# Autodesk Inventor assembly: SP40-10 MARCO HOJA CORREDERA 1131x695
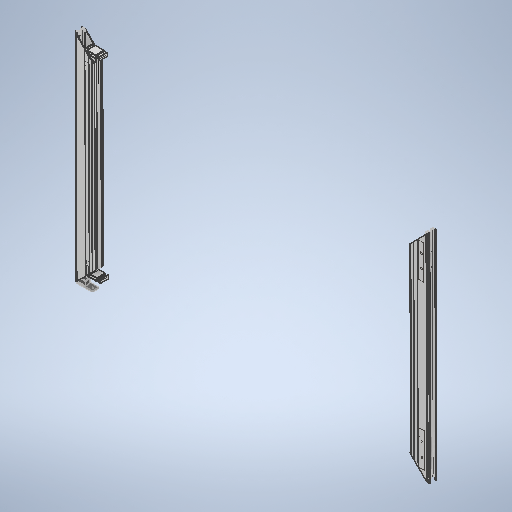
[picture p0: Inventor's stored thumbnail of the model, 512x512]
Saved by Autodesk Inventor 2025 (Build 290162000, 162)
## iProperties
Created: 2026-02-17
Part Number: SP40-10 MARCO HOJA CORREDERA 1131x695
Document SubType Name: Assembly
Designer: Frank
Author: Frank
## Documents named in this file (29)
- C:\Users\Frank\OneDrive\CARPINTERIA ALUMINIO\PUERTAS Y VENTANAS\VENTANAS\VENTANAS\ENSAMBLES\HOJA CORREDERA SP40-10 EXT 1400x1200 - DERECHA TRASERA.iam
- C:\Users\Frank\OneDrive\CARPINTERIA ALUMINIO\PUERTAS Y VENTANAS\VENTANAS\VENTANAS\PIEZAS\HOJA CORREDERA SP40-10 EXT 1400x1200\SP40-10 HOJA CORREDERA 1131 mm.ipt
- C:\Users\Frank\OneDrive\CARPINTERIA ALUMINIO\PUERTAS Y VENTANAS\VENTANAS\VENTANAS\PIEZAS\HOJA CORREDERA SP40-10 EXT 1400x1200\SP40-10 HOJA CORREDERA 695 mm.ipt
- C:\Users\Frank\OneDrive\CARPINTERIA ALUMINIO\PUERTAS Y VENTANAS\VENTANAS\VENTANAS\PIEZAS\HOJA CORREDERA SP40-10 EXT 1400x1200\SP40-10 HOJA CORREDERA 695 mm_MIR.ipt
- C:\Users\Frank\OneDrive\CARPINTERIA ALUMINIO\PUERTAS Y VENTANAS\VENTANAS\VENTANAS\PIEZAS\HOJA CORREDERA SP40-10 EXT 1400x1200\SP40-10 HOJA CORREDERA 1131 mm_MIR.ipt
- C:\Users\Frank\OneDrive\CARPINTERIA ALUMINIO\PUERTAS Y VENTANAS\VENTANAS\VENTANAS\PIEZAS\HOJA CORREDERA SP40-10 EXT 1400x1200\BRA-12 ESCUADRA UNIÓN 45 10 mm.ipt
- C:\Users\Frank\OneDrive\CARPINTERIA ALUMINIO\PUERTAS Y VENTANAS\VENTANAS\VENTANAS\PIEZAS\HOJA CORREDERA SP40-10 EXT 1400x1200\BRA-12 ESCUADRA UNIÓN 45 10 mm_MIR.ipt
- C:\Users\Frank\OneDrive\CARPINTERIA ALUMINIO\PUERTAS Y VENTANAS\VENTANAS\VENTANAS\PIEZAS\HOJA CORREDERA SP40-10 EXT 1400x1200\BRA-12 ESCUADRA UNIÓN 45 10 mm_MIR1.ipt
- C:\Users\Frank\OneDrive\CARPINTERIA ALUMINIO\PUERTAS Y VENTANAS\VENTANAS\VENTANAS\PIEZAS\HOJA CORREDERA SP40-10 EXT 1400x1200\BRA-12 ESCUADRA UNIÓN 45 10 mm_MIR2.ipt
- C:\Users\Frank\OneDrive\CARPINTERIA ALUMINIO\PUERTAS Y VENTANAS\VENTANAS\VENTANAS\PIEZAS\HOJA CORREDERA SP40-10 EXT 1400x1200\SP40-10 JUNTA INT 1025 mm.ipt
- C:\Users\Frank\OneDrive\CARPINTERIA ALUMINIO\PUERTAS Y VENTANAS\VENTANAS\VENTANAS\PIEZAS\HOJA CORREDERA SP40-10 EXT 1400x1200\SP40-10 JUNTA INT 1025 mm_MIR.ipt
- C:\Users\Frank\OneDrive\CARPINTERIA ALUMINIO\PUERTAS Y VENTANAS\VENTANAS\VENTANAS\PIEZAS\HOJA CORREDERA SP40-10 EXT 1400x1200\SP40-10 JUNTA INT 589 mm.ipt
- C:\Users\Frank\OneDrive\CARPINTERIA ALUMINIO\PUERTAS Y VENTANAS\VENTANAS\VENTANAS\PIEZAS\HOJA CORREDERA SP40-10 EXT 1400x1200\SP40-10 JUNTA INT 589 mm_MIR.ipt
- C:\Users\Frank\OneDrive\CARPINTERIA ALUMINIO\PUERTAS Y VENTANAS\VENTANAS\VENTANAS\PIEZAS\HOJA CORREDERA SP40-10 EXT 1400x1200\PLANCHA DE CRISTAL TRANSPARENTE 1033x597.ipt
- C:\Users\Frank\OneDrive\CARPINTERIA ALUMINIO\PUERTAS Y VENTANAS\VENTANAS\VENTANAS\PIEZAS\HOJA CORREDERA SP40-10 EXT 1400x1200\SP40-10 JUNTA INT CRISTAL 1023 mm.ipt
- C:\Users\Frank\OneDrive\CARPINTERIA ALUMINIO\PUERTAS Y VENTANAS\VENTANAS\VENTANAS\PIEZAS\HOJA CORREDERA SP40-10 EXT 1400x1200\SP40-10 JUNTA INT CRISTAL 1023 mm_MIR.ipt
- C:\Users\Frank\OneDrive\CARPINTERIA ALUMINIO\PUERTAS Y VENTANAS\VENTANAS\VENTANAS\PIEZAS\HOJA CORREDERA SP40-10 EXT 1400x1200\SP40-10 JUNTA INT CRISTAL 587 mm.ipt
- C:\Users\Frank\OneDrive\CARPINTERIA ALUMINIO\PUERTAS Y VENTANAS\VENTANAS\VENTANAS\PIEZAS\HOJA CORREDERA SP40-10 EXT 1400x1200\SP40-10 JUNTA INT CRISTAL 587 mm_MIR.ipt
- C:\Users\Frank\OneDrive\CARPINTERIA ALUMINIO\PUERTAS Y VENTANAS\VENTANAS\VENTANAS\PIEZAS\HOJA CORREDERA SP40-10 EXT 1400x1200\SP40-10 JUNTA DE FELPA 693 mm.ipt
- C:\Users\Frank\OneDrive\CARPINTERIA ALUMINIO\PUERTAS Y VENTANAS\VENTANAS\VENTANAS\PIEZAS\HOJA CORREDERA SP40-10 EXT 1400x1200\SP40-10 JUNTA DE FELPA 693 mm_MIR1.ipt
- C:\Users\Frank\OneDrive\CARPINTERIA ALUMINIO\PUERTAS Y VENTANAS\VENTANAS\VENTANAS\PIEZAS\HOJA CORREDERA SP40-10 EXT 1400x1200\SP40-10 JUNTA DE FELPA 1118 mm.ipt
- C:\Users\Frank\OneDrive\CARPINTERIA ALUMINIO\PUERTAS Y VENTANAS\VENTANAS\VENTANAS\PIEZAS\HOJA CORREDERA SP40-10 EXT 1400x1200\SP40-10 JUNTA DE FELPA 1118 mm_MIR3.ipt
- C:\Users\Frank\OneDrive\CARPINTERIA ALUMINIO\PUERTAS Y VENTANAS\VENTANAS\VENTANAS\PIEZAS\HOJA CORREDERA SP40-10 EXT 1400x1200\SP40-11 TAPETA - ENCUENTRO HOJA CORREDERA 695 mm.ipt
- C:\Users\Frank\OneDrive\CARPINTERIA ALUMINIO\PUERTAS Y VENTANAS\ACCESORIOS\TAPONES PLASTICOS\PLU-45 TAPÓN ENCUENTRO CORREDERA (1).ipt
- C:\Users\Frank\OneDrive\CARPINTERIA ALUMINIO\PUERTAS Y VENTANAS\ACCESORIOS\TAPONES PLASTICOS\PLU-45 TAPÓN ENCUENTRO CORREDERA (2).ipt
- C:\Users\Frank\OneDrive\CARPINTERIA ALUMINIO\PUERTAS Y VENTANAS\VENTANAS\VENTANAS\PIEZAS\HOJA CORREDERA SP40-10 EXT 1400x1200\SP40-11 JUNTA DE FELPA PARA ENCUENTRO HOJA CORREDERA 695 mm.ipt
- C:\Users\Frank\OneDrive\CARPINTERIA ALUMINIO\PUERTAS Y VENTANAS\VENTANAS\VENTANAS\PIEZAS\HOJA CORREDERA SP40-10 EXT 1400x1200\SP40-10 JUNTA DE FELPA 693 mm_MIR3.ipt
- C:\Users\Frank\OneDrive\CARPINTERIA ALUMINIO\PUERTAS Y VENTANAS\VENTANAS\VENTANAS\PIEZAS\HOJA CORREDERA SP40-10 EXT 1400x1200\SP40-10 JUNTA DE FELPA 693 mm_MIR1_MIR.ipt
- C:\Users\Frank\OneDrive\CARPINTERIA ALUMINIO\PUERTAS Y VENTANAS\ACCESORIOS\RODAMIENTO\WHE-012 RODAMIENTO.iam
## Components (29 placed, 28 different names)
1. SP40-10 HOJA CORREDERA 1131 mm:1 — Coincidencia:1, Coincidencia:21, Coincidencia:23, Coincidencia:24, Coincidencia:25, Coincidencia:33, Coincidencia:34, Coincidencia:43, Coincidencia:44, Coincidencia:46, Coincidencia:47, Nivelación:5, Nivelación:11, Coincidencia:52, Coincidencia:53, Coincidencia:74, Coincidencia:75, Coincidencia:76, Coincidencia:93
2. SP40-10 HOJA CORREDERA 695 mm:1 — Coincidencia:17, Coincidencia:18, Coincidencia:19, Coincidencia:22, Coincidencia:29, Coincidencia:45, Coincidencia:50, Nivelación:9, Nivelación:10, Nivelación:12, Coincidencia:54, Coincidencia:55, Coincidencia:66, Coincidencia:67, Coincidencia:68, Coincidencia:69, Simetría:1, Coincidencia:91, Coincidencia:92, Coincidencia:94, Coincidencia:95, Coincidencia:96
3. SP40-10 HOJA CORREDERA 695 mm_MIR:1 — Coincidencia:14, Coincidencia:15, Coincidencia:16, Coincidencia:26, Coincidencia:30, Coincidencia:31, Coincidencia:33, Coincidencia:34, Coincidencia:41, Coincidencia:49, Nivelación:7, Nivelación:8, Nivelación:13, Coincidencia:56, Simetría:1, Nivelación:19, Nivelación:20, Coincidencia:87, Coincidencia:88, Coincidencia:89, Coincidencia:90
4. SP40-10 HOJA CORREDERA 1131 mm_MIR:1 — Coincidencia:14, Coincidencia:15, Coincidencia:16, Coincidencia:17, Coincidencia:18, Coincidencia:19, Coincidencia:27, Coincidencia:28, Coincidencia:32, Coincidencia:35, Coincidencia:36, Nivelación:6, Coincidencia:48, Coincidencia:51, Coincidencia:70, Coincidencia:71, Nivelación:17, Coincidencia:72, Coincidencia:73, Nivelación:21
5. BRA-12 ESCUADRA UNIÓN 45 10 mm:1 — Coincidencia:21, Coincidencia:22, Coincidencia:23
6. BRA-12 ESCUADRA UNIÓN 45 10 mm_MIR:1 — Coincidencia:24, Coincidencia:25, Coincidencia:26
7. BRA-12 ESCUADRA UNIÓN 45 10 mm_MIR1:1 — Coincidencia:27, Coincidencia:28, Coincidencia:29
8. BRA-12 ESCUADRA UNIÓN 45 10 mm_MIR2:1 — Coincidencia:30, Coincidencia:31, Coincidencia:32
9. SP40-10 JUNTA INT 1025 mm:1 — Coincidencia:35, Coincidencia:36, Coincidencia:51
10. SP40-10 JUNTA INT 1025 mm_MIR:1 — Nivelación:11, Coincidencia:52, Coincidencia:53
11. SP40-10 JUNTA INT 589 mm:1 — Nivelación:12, Coincidencia:54, Coincidencia:55
12. SP40-10 JUNTA INT 589 mm_MIR:1 — Coincidencia:41, Nivelación:13, Coincidencia:56
13. PLANCHA DE CRISTAL TRANSPARENTE 1033x597:1 — Coincidencia:43, Coincidencia:44, Coincidencia:45
14. SP40-10 JUNTA INT CRISTAL 1023 mm:1 — Coincidencia:46, Coincidencia:47, Nivelación:5
15. SP40-10 JUNTA INT CRISTAL 1023 mm_MIR:1 — Nivelación:6, Coincidencia:48
16. SP40-10 JUNTA INT CRISTAL 587 mm:1 — Coincidencia:49, Nivelación:7, Nivelación:8
17. SP40-10 JUNTA INT CRISTAL 587 mm_MIR:1 — Coincidencia:50, Nivelación:9, Nivelación:10
18. SP40-10 JUNTA DE FELPA 693 mm:1 — Coincidencia:66, Coincidencia:67, Coincidencia:85
19. SP40-10 JUNTA DE FELPA 693 mm_MIR1:1 — Coincidencia:68, Coincidencia:69, Coincidencia:86
20. SP40-10 JUNTA DE FELPA 1118 mm:1 — Coincidencia:70, Coincidencia:71, Nivelación:21
21. SP40-10 JUNTA DE FELPA 1118 mm_MIR3:1 — Nivelación:17, Coincidencia:72, Coincidencia:73
22. SP40-11 TAPETA - ENCUENTRO HOJA CORREDERA 695 mm:1 — Coincidencia:74, Coincidencia:75, Coincidencia:76, Coincidencia:77, Coincidencia:78, Coincidencia:79, Coincidencia:80, Coincidencia:81, Coincidencia:82, Coincidencia:83, Coincidencia:84, Nivelación:18
23. PLU-45 TAPÓN ENCUENTRO CORREDERA (1):1 — Coincidencia:77, Coincidencia:78, Coincidencia:79, Coincidencia:85, Coincidencia:86
24. PLU-45 TAPÓN ENCUENTRO CORREDERA (2):1 — Coincidencia:80, Coincidencia:81, Coincidencia:82
25. SP40-11 JUNTA DE FELPA PARA ENCUENTRO HOJA CORREDERA 695 mm:1 — Coincidencia:83, Coincidencia:84, Nivelación:18
26. SP40-10 JUNTA DE FELPA 693 mm_MIR3:1 — Nivelación:19, Coincidencia:89, Coincidencia:90
27. SP40-10 JUNTA DE FELPA 693 mm_MIR1_MIR:1 — Nivelación:20, Coincidencia:87, Coincidencia:88
28. WHE-012 RODAMIENTO:1 [sub-assembly] — Coincidencia:91, Coincidencia:92, Coincidencia:93
29. WHE-012 RODAMIENTO:2 [sub-assembly] — Coincidencia:94, Coincidencia:95, Coincidencia:96
## Relationships (84: Mate 69, Flush 14, Symmetry 1)
- Coincidencia:1 [Mate]: SP40-10 HOJA CORREDERA 1131 mm:1
- Coincidencia:14 [Mate]: SP40-10 HOJA CORREDERA 695 mm_MIR:1 ↔ SP40-10 HOJA CORREDERA 1131 mm_MIR:1
- Coincidencia:15 [Mate]: SP40-10 HOJA CORREDERA 695 mm_MIR:1 ↔ SP40-10 HOJA CORREDERA 1131 mm_MIR:1
- Coincidencia:16 [Mate]: SP40-10 HOJA CORREDERA 695 mm_MIR:1 ↔ SP40-10 HOJA CORREDERA 1131 mm_MIR:1
- Coincidencia:17 [Mate]: SP40-10 HOJA CORREDERA 695 mm:1 ↔ SP40-10 HOJA CORREDERA 1131 mm_MIR:1
- Coincidencia:18 [Mate]: SP40-10 HOJA CORREDERA 695 mm:1 ↔ SP40-10 HOJA CORREDERA 1131 mm_MIR:1
- Coincidencia:19 [Mate]: SP40-10 HOJA CORREDERA 695 mm:1 ↔ SP40-10 HOJA CORREDERA 1131 mm_MIR:1
- Coincidencia:21 [Mate] (0.6 mm): SP40-10 HOJA CORREDERA 1131 mm:1 ↔ BRA-12 ESCUADRA UNIÓN 45 10 mm:1
- Coincidencia:22 [Mate]: SP40-10 HOJA CORREDERA 695 mm:1 ↔ BRA-12 ESCUADRA UNIÓN 45 10 mm:1
- Coincidencia:23 [Mate]: SP40-10 HOJA CORREDERA 1131 mm:1 ↔ BRA-12 ESCUADRA UNIÓN 45 10 mm:1
- Coincidencia:24 [Mate] (0.6 mm): SP40-10 HOJA CORREDERA 1131 mm:1 ↔ BRA-12 ESCUADRA UNIÓN 45 10 mm_MIR:1
- Coincidencia:25 [Mate]: SP40-10 HOJA CORREDERA 1131 mm:1 ↔ BRA-12 ESCUADRA UNIÓN 45 10 mm_MIR:1
- Coincidencia:26 [Mate]: SP40-10 HOJA CORREDERA 695 mm_MIR:1 ↔ BRA-12 ESCUADRA UNIÓN 45 10 mm_MIR:1
- Coincidencia:27 [Mate] (0.6 mm): SP40-10 HOJA CORREDERA 1131 mm_MIR:1 ↔ BRA-12 ESCUADRA UNIÓN 45 10 mm_MIR1:1
- Coincidencia:28 [Mate]: SP40-10 HOJA CORREDERA 1131 mm_MIR:1 ↔ BRA-12 ESCUADRA UNIÓN 45 10 mm_MIR1:1
- Coincidencia:29 [Mate]: SP40-10 HOJA CORREDERA 695 mm:1 ↔ BRA-12 ESCUADRA UNIÓN 45 10 mm_MIR1:1
- Coincidencia:30 [Mate] (0.6 mm): SP40-10 HOJA CORREDERA 695 mm_MIR:1 ↔ BRA-12 ESCUADRA UNIÓN 45 10 mm_MIR2:1
- Coincidencia:31 [Mate]: SP40-10 HOJA CORREDERA 695 mm_MIR:1 ↔ BRA-12 ESCUADRA UNIÓN 45 10 mm_MIR2:1
- Coincidencia:32 [Mate]: SP40-10 HOJA CORREDERA 1131 mm_MIR:1 ↔ BRA-12 ESCUADRA UNIÓN 45 10 mm_MIR2:1
- Coincidencia:33 [Mate]: SP40-10 HOJA CORREDERA 1131 mm:1 ↔ SP40-10 HOJA CORREDERA 695 mm_MIR:1
- Coincidencia:34 [Mate]: SP40-10 HOJA CORREDERA 1131 mm:1 ↔ SP40-10 HOJA CORREDERA 695 mm_MIR:1
- Coincidencia:35 [Mate]: SP40-10 HOJA CORREDERA 1131 mm_MIR:1 ↔ SP40-10 JUNTA INT 1025 mm:1
- Coincidencia:36 [Mate]: SP40-10 HOJA CORREDERA 1131 mm_MIR:1 ↔ SP40-10 JUNTA INT 1025 mm:1
- Coincidencia:41 [Mate]: SP40-10 HOJA CORREDERA 695 mm_MIR:1 ↔ SP40-10 JUNTA INT 589 mm_MIR:1
- Coincidencia:43 [Mate] (2.45 mm): SP40-10 HOJA CORREDERA 1131 mm:1 ↔ PLANCHA DE CRISTAL TRANSPARENTE 1033x597:1
- Coincidencia:44 [Mate] (4 mm): SP40-10 HOJA CORREDERA 1131 mm:1 ↔ PLANCHA DE CRISTAL TRANSPARENTE 1033x597:1
- Coincidencia:45 [Mate] (2.5 mm): SP40-10 HOJA CORREDERA 695 mm:1 ↔ PLANCHA DE CRISTAL TRANSPARENTE 1033x597:1
- Coincidencia:46 [Mate]: SP40-10 HOJA CORREDERA 1131 mm:1 ↔ SP40-10 JUNTA INT CRISTAL 1023 mm:1
- Coincidencia:47 [Mate]: SP40-10 HOJA CORREDERA 1131 mm:1 ↔ SP40-10 JUNTA INT CRISTAL 1023 mm:1
- Nivelación:5 [Flush]: SP40-10 HOJA CORREDERA 1131 mm:1 ↔ SP40-10 JUNTA INT CRISTAL 1023 mm:1
- Nivelación:6 [Flush]: SP40-10 HOJA CORREDERA 1131 mm_MIR:1 ↔ SP40-10 JUNTA INT CRISTAL 1023 mm_MIR:1
- Coincidencia:48 [Mate]: SP40-10 HOJA CORREDERA 1131 mm_MIR:1 ↔ SP40-10 JUNTA INT CRISTAL 1023 mm_MIR:1
- Coincidencia:49 [Mate]: SP40-10 HOJA CORREDERA 695 mm_MIR:1 ↔ SP40-10 JUNTA INT CRISTAL 587 mm:1
- Nivelación:7 [Flush]: SP40-10 HOJA CORREDERA 695 mm_MIR:1 ↔ SP40-10 JUNTA INT CRISTAL 587 mm:1
- Nivelación:8 [Flush]: SP40-10 HOJA CORREDERA 695 mm_MIR:1 ↔ SP40-10 JUNTA INT CRISTAL 587 mm:1
- Coincidencia:50 [Mate]: SP40-10 HOJA CORREDERA 695 mm:1 ↔ SP40-10 JUNTA INT CRISTAL 587 mm_MIR:1
- Nivelación:9 [Flush]: SP40-10 HOJA CORREDERA 695 mm:1 ↔ SP40-10 JUNTA INT CRISTAL 587 mm_MIR:1
- Nivelación:10 [Flush]: SP40-10 HOJA CORREDERA 695 mm:1 ↔ SP40-10 JUNTA INT CRISTAL 587 mm_MIR:1
- Coincidencia:51 [Mate]: SP40-10 HOJA CORREDERA 1131 mm_MIR:1 ↔ SP40-10 JUNTA INT 1025 mm:1
- Nivelación:11 [Flush]: SP40-10 HOJA CORREDERA 1131 mm:1 ↔ SP40-10 JUNTA INT 1025 mm_MIR:1
- Coincidencia:52 [Mate]: SP40-10 HOJA CORREDERA 1131 mm:1 ↔ SP40-10 JUNTA INT 1025 mm_MIR:1
- Coincidencia:53 [Mate]: SP40-10 HOJA CORREDERA 1131 mm:1 ↔ SP40-10 JUNTA INT 1025 mm_MIR:1
- Nivelación:12 [Flush]: SP40-10 HOJA CORREDERA 695 mm:1 ↔ SP40-10 JUNTA INT 589 mm:1
- Coincidencia:54 [Mate]: SP40-10 HOJA CORREDERA 695 mm:1 ↔ SP40-10 JUNTA INT 589 mm:1
- Coincidencia:55 [Mate]: SP40-10 HOJA CORREDERA 695 mm:1 ↔ SP40-10 JUNTA INT 589 mm:1
- Nivelación:13 [Flush]: SP40-10 HOJA CORREDERA 695 mm_MIR:1 ↔ SP40-10 JUNTA INT 589 mm_MIR:1
- Coincidencia:56 [Mate]: SP40-10 HOJA CORREDERA 695 mm_MIR:1 ↔ SP40-10 JUNTA INT 589 mm_MIR:1
- Coincidencia:66 [Mate]: SP40-10 HOJA CORREDERA 695 mm:1 ↔ SP40-10 JUNTA DE FELPA 693 mm:1
- Coincidencia:67 [Mate]: SP40-10 HOJA CORREDERA 695 mm:1 ↔ SP40-10 JUNTA DE FELPA 693 mm:1
- Coincidencia:68 [Mate]: SP40-10 HOJA CORREDERA 695 mm:1 ↔ SP40-10 JUNTA DE FELPA 693 mm_MIR1:1
- Coincidencia:69 [Mate]: SP40-10 HOJA CORREDERA 695 mm:1 ↔ SP40-10 JUNTA DE FELPA 693 mm_MIR1:1
- Coincidencia:70 [Mate]: SP40-10 HOJA CORREDERA 1131 mm_MIR:1 ↔ SP40-10 JUNTA DE FELPA 1118 mm:1
- Coincidencia:71 [Mate]: SP40-10 HOJA CORREDERA 1131 mm_MIR:1 ↔ SP40-10 JUNTA DE FELPA 1118 mm:1
- Nivelación:17 [Flush]: SP40-10 HOJA CORREDERA 1131 mm_MIR:1 ↔ SP40-10 JUNTA DE FELPA 1118 mm_MIR3:1
- Coincidencia:72 [Mate]: SP40-10 HOJA CORREDERA 1131 mm_MIR:1 ↔ SP40-10 JUNTA DE FELPA 1118 mm_MIR3:1
- Coincidencia:73 [Mate]: SP40-10 HOJA CORREDERA 1131 mm_MIR:1 ↔ SP40-10 JUNTA DE FELPA 1118 mm_MIR3:1
- Coincidencia:74 [Mate]: SP40-10 HOJA CORREDERA 1131 mm:1 ↔ SP40-11 TAPETA - ENCUENTRO HOJA CORREDERA 695 mm:1
- Coincidencia:75 [Mate]: SP40-10 HOJA CORREDERA 1131 mm:1 ↔ SP40-11 TAPETA - ENCUENTRO HOJA CORREDERA 695 mm:1
- Coincidencia:76 [Mate]: SP40-10 HOJA CORREDERA 1131 mm:1 ↔ SP40-11 TAPETA - ENCUENTRO HOJA CORREDERA 695 mm:1
- Coincidencia:77 [Mate]: SP40-11 TAPETA - ENCUENTRO HOJA CORREDERA 695 mm:1 ↔ PLU-45 TAPÓN ENCUENTRO CORREDERA (1):1
- Coincidencia:78 [Mate]: SP40-11 TAPETA - ENCUENTRO HOJA CORREDERA 695 mm:1 ↔ PLU-45 TAPÓN ENCUENTRO CORREDERA (1):1
- Coincidencia:79 [Mate]: SP40-11 TAPETA - ENCUENTRO HOJA CORREDERA 695 mm:1 ↔ PLU-45 TAPÓN ENCUENTRO CORREDERA (1):1
- Coincidencia:80 [Mate]: SP40-11 TAPETA - ENCUENTRO HOJA CORREDERA 695 mm:1 ↔ PLU-45 TAPÓN ENCUENTRO CORREDERA (2):1
- Coincidencia:81 [Mate]: SP40-11 TAPETA - ENCUENTRO HOJA CORREDERA 695 mm:1 ↔ PLU-45 TAPÓN ENCUENTRO CORREDERA (2):1
- Coincidencia:82 [Mate]: SP40-11 TAPETA - ENCUENTRO HOJA CORREDERA 695 mm:1 ↔ PLU-45 TAPÓN ENCUENTRO CORREDERA (2):1
- Coincidencia:83 [Mate]: SP40-11 TAPETA - ENCUENTRO HOJA CORREDERA 695 mm:1 ↔ SP40-11 JUNTA DE FELPA PARA ENCUENTRO HOJA CORREDERA 695 mm:1
- Coincidencia:84 [Mate]: SP40-11 TAPETA - ENCUENTRO HOJA CORREDERA 695 mm:1 ↔ SP40-11 JUNTA DE FELPA PARA ENCUENTRO HOJA CORREDERA 695 mm:1
- Nivelación:18 [Flush]: SP40-11 TAPETA - ENCUENTRO HOJA CORREDERA 695 mm:1 ↔ SP40-11 JUNTA DE FELPA PARA ENCUENTRO HOJA CORREDERA 695 mm:1
- Coincidencia:85 [Mate]: SP40-10 JUNTA DE FELPA 693 mm:1 ↔ PLU-45 TAPÓN ENCUENTRO CORREDERA (1):1
- Coincidencia:86 [Mate]: SP40-10 JUNTA DE FELPA 693 mm_MIR1:1 ↔ PLU-45 TAPÓN ENCUENTRO CORREDERA (1):1
- Simetría:1 [Symmetry]: SP40-10 HOJA CORREDERA 695 mm:1 ↔ SP40-10 HOJA CORREDERA 695 mm_MIR:1
- Nivelación:19 [Flush]: SP40-10 HOJA CORREDERA 695 mm_MIR:1 ↔ SP40-10 JUNTA DE FELPA 693 mm_MIR3:1
- Nivelación:20 [Flush]: SP40-10 HOJA CORREDERA 695 mm_MIR:1 ↔ SP40-10 JUNTA DE FELPA 693 mm_MIR1_MIR:1
- Coincidencia:87 [Mate]: SP40-10 HOJA CORREDERA 695 mm_MIR:1 ↔ SP40-10 JUNTA DE FELPA 693 mm_MIR1_MIR:1
- Coincidencia:88 [Mate]: SP40-10 HOJA CORREDERA 695 mm_MIR:1 ↔ SP40-10 JUNTA DE FELPA 693 mm_MIR1_MIR:1
- Coincidencia:89 [Mate]: SP40-10 HOJA CORREDERA 695 mm_MIR:1 ↔ SP40-10 JUNTA DE FELPA 693 mm_MIR3:1
- Coincidencia:90 [Mate]: SP40-10 HOJA CORREDERA 695 mm_MIR:1 ↔ SP40-10 JUNTA DE FELPA 693 mm_MIR3:1
- Nivelación:21 [Flush]: SP40-10 HOJA CORREDERA 1131 mm_MIR:1 ↔ SP40-10 JUNTA DE FELPA 1118 mm:1
- Coincidencia:91 [Mate]: SP40-10 HOJA CORREDERA 695 mm:1 ↔ WHE-012 RODAMIENTO:1
- Coincidencia:92 [Mate]: SP40-10 HOJA CORREDERA 695 mm:1 ↔ WHE-012 RODAMIENTO:1
- Coincidencia:93 [Mate]: SP40-10 HOJA CORREDERA 1131 mm:1 ↔ WHE-012 RODAMIENTO:1
- Coincidencia:94 [Mate]: SP40-10 HOJA CORREDERA 695 mm:1 ↔ WHE-012 RODAMIENTO:2
- Coincidencia:95 [Mate]: SP40-10 HOJA CORREDERA 695 mm:1 ↔ WHE-012 RODAMIENTO:2
- Coincidencia:96 [Mate]: SP40-10 HOJA CORREDERA 695 mm:1 ↔ WHE-012 RODAMIENTO:2
